# Autodesk Inventor assembly: ArmTruss_MIR
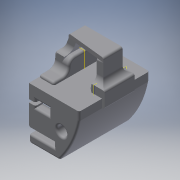
[picture p0: Inventor's stored thumbnail of the model, 180x180]
Saved by Autodesk Inventor 2018 (Build 220112000, 112)
## iProperties
Created: 2017-12-31
Part Number: ArmTruss_MIR
Document SubType Name: Assembly
Designer: reide
Author: reide
## Documents named in this file (4)
- C:\Users\reide\OneDrive\Documents\Inventor\TSA\2019\Animatronics\Glyptodon\Glyptodon Work\Arms\ArmTruss_MIR.iam
- C:\Users\reide\OneDrive\Documents\Inventor\TSA\2019\Animatronics\Glyptodon\Glyptodon Work\Arms\newShoulder_MIR1.ipt
- C:\Users\reide\OneDrive\Documents\Inventor\TSA\2019\Animatronics\Glyptodon\Glyptodon Work\Arms\straightBar_MIR1.ipt
- C:\Users\reide\OneDrive\Documents\Inventor\TSA\2019\Animatronics\Glyptodon\Glyptodon Work\Arms\bottomARM_MIR1.ipt
## Components (3 placed, 3 different names)
1. newShoulder_MIR1:1 — Flush:4, Flush:3, Mate:5, Mate:6, Mate:7
2. bottomARM_MIR1:1 — Flush:4, Flush:3, Mate:5, Flush:5
3. straightBar_MIR1:2 — Mate:6, Mate:7, Flush:5
## Relationships (6: Flush 3, Mate 3)
- Flush:4: newShoulder_MIR1:1 ↔ bottomARM_MIR1:1
- Flush:3: newShoulder_MIR1:1 ↔ bottomARM_MIR1:1
- Mate:5: newShoulder_MIR1:1 ↔ bottomARM_MIR1:1
- Mate:6: newShoulder_MIR1:1 ↔ straightBar_MIR1:2
- Mate:7: newShoulder_MIR1:1 ↔ straightBar_MIR1:2
- Flush:5: bottomARM_MIR1:1 ↔ straightBar_MIR1:2
